# Autodesk Inventor assembly: FullField-ver6-1111-2021
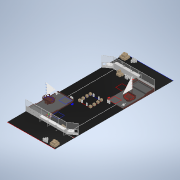
[picture p0: Inventor's stored thumbnail of the model, 180x180]
Saved by Autodesk Inventor 2021 (Build 250183000, 183)
## iProperties
Created: 2021-02-23
Part Number: FullField-ver6-1111-2021
Document SubType Name: Assembly
Designer: CMurray
Author: CMurray
## Documents named in this file (30)
- F:\PHRC CADD 2021\2021 Game Design Challenge\Full Field\Final Assembly\FullField-ver6-1111-2021.iam
- F:\PHRC CADD 2021\2021 Game Design Challenge\Full Field\Parts\FieldFloor-ver1-1111-2021.ipt
- F:\PHRC CADD 2021\2021 Game Design Challenge\Full Field\Parts\Tape\Tape.ipt
- F:\PHRC CADD 2021\2021 Game Design Challenge\Full Field\Parts\Tape\RedAllianceTape-ver1-1111-2021.ipt
- F:\PHRC CADD 2021\2021 Game Design Challenge\Full Field\Parts\Tape\BlueAllianceTape-ver1-1111-2021.ipt
- F:\PHRC CADD 2021\2021 Game Design Challenge\Player Station\Assemblies\DriverStation-ver2-1111-2021.iam
- F:\PHRC CADD 2021\2021 Game Design Challenge\Crow's Nest\Assemblies\CrowsNestFinal-ver3-1111-2021.iam
- F:\PHRC CADD 2021\2021 Game Design Challenge\Main Ship\RedShip-ver1-1111-2021.ipt
- F:\PHRC CADD 2021\2021 Game Design Challenge\Crow's Nest\Parts\Capstan\test.ipt
- F:\PHRC CADD 2021\2021 Game Design Challenge\Crow's Nest\Parts\Capstan\CapTop-ver1-1111-2021.ipt
- F:\PHRC CADD 2021\2021 Game Design Challenge\Crow's Nest\Parts\Capstan\FullSailCapstan-ver2-1111-2021.iam
- F:\PHRC CADD 2021\2021 Game Design Challenge\Full Field\Parts\Tape\Tape2.ipt
- F:\PHRC CADD 2021\2021 Game Design Challenge\Main Ship\BlueShip-ver1-1111-2021.ipt
- F:\PHRC CADD 2021\2021 Game Design Challenge\Crow's Nest\Assemblies\BlueCrowsNestFinal-ver1-1111-2021.iam
- F:\PHRC CADD 2021\2021 Game Design Challenge\Misc\cargoPrototype.ipt
- F:\PHRC CADD 2021\2021 Game Design Challenge\Full Field\Parts\Tape\MidSquareFull.iam
- F:\PHRC CADD 2021\2021 Game Design Challenge\Treasure Chest\PTreasureChestFinal-ver1-1111-2021.ipt
- F:\PHRC CADD 2021\2021 Game Design Challenge\Full Field\Parts\Tape\RedAllianceTape-ver2-1111-2021.ipt
- F:\PHRC CADD 2021\2021 Game Design Challenge\Full Field\Parts\Tape\BlueAllianceTape-ver2-1111-2021.ipt
- F:\PHRC CADD 2021\2021 Game Design Challenge\Anchor\CapstanBottom-ver1-1111-2021.ipt
- F:\PHRC CADD 2021\2021 Game Design Challenge\Anchor\CapstanTop-ver1-1111-2021.ipt
- F:\PHRC CADD 2021\2021 Game Design Challenge\Misc\WaterJug-ver1-1111-2021.ipt
- F:\PHRC CADD 2021\2021 Game Design Challenge\Treasure Chest\BlueMapContainer-ver1-1111-2021.ipt
- F:\PHRC CADD 2021\2021 Game Design Challenge\Treasure Chest\RedMapContainer-ver1-1111-2021.ipt
- F:\PHRC CADD 2021\2021 Game Design Challenge\Full Field\Parts\Tape\ParkingTapeBlueFull.iam
- F:\PHRC CADD 2021\2021 Game Design Challenge\Full Field\Parts\Tape\CrowsNestTapeBlue.ipt
- F:\PHRC CADD 2021\2021 Game Design Challenge\Full Field\Parts\Tape\CrowsNestTapeRed.ipt
- F:\PHRC CADD 2021\2021 Game Design Challenge\Full Field\Parts\Tape\ParkingTapeRedFull.iam
- F:\PHRC CADD 2021\2021 Game Design Challenge\Anchor\CapBottomwChain.iam
- F:\PHRC CADD 2021\2021 Game Design Challenge\Anchor\anchorPlaceholder.ipt
## Components (117 placed, 29 different names)
1. FieldFloor-ver1-1111-2021:1 — Flush:1, Flush:2, Mate:1, Mate:3, Mate:10, Flush:10, Mate:14, Flush:12, Mate:32, Mate:34, Mate:51, Flush:24, Mate:53, Flush:25, Mate:63, Mate:75, Mate:76, Mate:88, Flush:26, Mate:104, Mate:105, Mate:106, Mate:107, Mate:108, Mate:109, Mate:110, Mate:111, Mate:112, Flush:30, Mate:121, Mate:122, Mate:131, Mate:138, Mate:139, Mate:140, Mate:141, Mate:142, Mate:143, Mate:146, Mate:147, Mate:148, Mate:149, Mate:150, Mate:156, Mate:157, Mate:158, Mate:159, Mate:160, Mate:161, Mate:173
2. FieldFloor-ver1-1111-2021:2 — Flush:1, Flush:2, Mate:1, Mate:2, Flush:3, Flush:4, Flush:5, Flush:6, Mate:8, Flush:9, Mate:12, Flush:11, Flush:19, Mate:36, Flush:20, Mate:49, Flush:23, Mate:62, Mate:72, Mate:77, Mate:78, Mate:79, Mate:80, Mate:83, Mate:85, Flush:27, Mate:89, Flush:28, Flush:29, Mate:90, Mate:91, Mate:92, Mate:93, Mate:94, Mate:95, Mate:96, Mate:97, Mate:98, Mate:123, Mate:124, Mate:125, Mate:126, Mate:127, Mate:128, Mate:129, Mate:130, Mate:132, Mate:133, Mate:134, Mate:135, Mate:137, Mate:144, Mate:152, Mate:153, Mate:154, Mate:155, Mate:162, Mate:163, Mate:164, Mate:165, Mate:167
3. WaterJug-ver1-1111-2021:1 — Mate:121
4. WaterJug-ver1-1111-2021:2 — Mate:122
5. WaterJug-ver1-1111-2021:3 — Mate:123
6. WaterJug-ver1-1111-2021:4 — Mate:124
7. WaterJug-ver1-1111-2021:5 — Mate:125
8. WaterJug-ver1-1111-2021:6 — Mate:126
9. WaterJug-ver1-1111-2021:7 — Mate:127
10. WaterJug-ver1-1111-2021:8 — Mate:128
11. WaterJug-ver1-1111-2021:9 — Mate:131
12. WaterJug-ver1-1111-2021:10 — Mate:129
13. WaterJug-ver1-1111-2021:11 — Mate:130
14. cargoPrototype:35 — Mate:137
15. cargoPrototype:36 — Mate:134
16. cargoPrototype:38 — Mate:133
17. cargoPrototype:39 — Mate:135, Mate:151
18. cargoPrototype:40 — Mate:132
19. cargoPrototype:41 — Mate:138
20. cargoPrototype:42 — Mate:142
21. cargoPrototype:43 — Mate:140
22. cargoPrototype:44 — Mate:141
23. cargoPrototype:45 — Mate:139, Mate:145
24. cargoPrototype:46 — Mate:145
25. BlueMapContainer-ver1-1111-2021:1 — Mate:143
26. RedMapContainer-ver1-1111-2021:1 — Mate:144
27. WaterJug-ver1-1111-2021:12 — Mate:146
28. WaterJug-ver1-1111-2021:13 — Mate:150
29. WaterJug-ver1-1111-2021:14 — Mate:147
30. WaterJug-ver1-1111-2021:15 — Mate:149
31. WaterJug-ver1-1111-2021:16 — Mate:148
32. cargoPrototype:47 — Mate:151
33. WaterJug-ver1-1111-2021:17 — Mate:152
34. WaterJug-ver1-1111-2021:18 — Mate:153
35. WaterJug-ver1-1111-2021:19 — Mate:154
36. WaterJug-ver1-1111-2021:20 — Mate:158
37. WaterJug-ver1-1111-2021:21 — Mate:156
38. WaterJug-ver1-1111-2021:22 — Mate:157
39. WaterJug-ver1-1111-2021:23 — Mate:159
40. WaterJug-ver1-1111-2021:24 — Mate:155
41. WaterJug-ver1-1111-2021:25 — Mate:162
42. WaterJug-ver1-1111-2021:26 — Mate:165
43. WaterJug-ver1-1111-2021:27 — Mate:164
44. WaterJug-ver1-1111-2021:28 — Mate:163
45. WaterJug-ver1-1111-2021:29 — Mate:160
46. WaterJug-ver1-1111-2021:30 — Mate:161
47. ParkingTapeBlueFull:1 [sub-assembly] — Mate:166
48. ParkingTapeBlueFull:2 [sub-assembly] — Mate:167
49. CrowsNestTapeBlue:1 — Mate:168, Mate:169
50. CrowsNestTapeRed:1 — Mate:170, Mate:171
51. ParkingTapeRedFull:1 [sub-assembly] — Mate:172
52. ParkingTapeRedFull:2 [sub-assembly] — Mate:173
53. CapBottomwChain:1 [sub-assembly] — Mate:174, Mate:175, Mate:176, Rotational:6
54. anchorPlaceholder:1
55. BlueAllianceTape-ver2-1111-2021:1 — Mate:89, Flush:28, Flush:29
56. RedAllianceTape-ver2-1111-2021:1 — Mate:88, Flush:26, Flush:27
57. MidSquareFull:1 [sub-assembly] — Mate:72, Mate:73, Mate:74
58. Tape2:1 — Mate:49, Flush:23, Mate:50
59. Tape2:2 — Mate:51, Flush:24, Mate:52, Mate:73
60. Tape:1 — Mate:2, Flush:3, Flush:4, Mate:9, Mate:11, Mate:33, Mate:50, Mate:74, Mate:87
61. Tape:2 — Mate:3, Flush:5, Flush:6, Mate:13, Mate:15, Mate:35, Mate:52, Mate:84
62. RedAllianceTape-ver1-1111-2021:1 — Mate:8, Flush:9, Mate:9
63. RedAllianceTape-ver1-1111-2021:2 — Mate:10, Flush:10, Mate:11
64. BlueAllianceTape-ver1-1111-2021:1 — Mate:12, Flush:11, Mate:13
65. BlueAllianceTape-ver1-1111-2021:2 — Mate:14, Flush:12, Mate:15
66. CapstanBottom-ver1-1111-2021:1 — Mate:117, Rotational:5, Flush:31, Flush:32
67. CapstanTop-ver1-1111-2021:1 — Rotational:5
68. CapTop-ver1-1111-2021:2
69. FullSailCapstan-ver2-1111-2021:3 [sub-assembly] — Rotational:4
70. test:2 — Mate:57, Mate:58, Mate:59, Rotational:4
71. BlueShip-ver1-1111-2021:1 — Mate:53, Mate:54, Flush:25, Mate:55, Mate:56, Mate:86, Mate:117, Flush:31, Flush:32
72. BlueCrowsNestFinal-ver1-1111-2021:1 [sub-assembly] — Mate:55, Mate:56, Mate:57, Mate:58, Mate:59, Mate:168, Mate:169
73. CapstanBottom-ver1-1111-2021:2 — Mate:118, Mate:119, Mate:120
74. CapstanTop-ver1-1111-2021:2 — Rotational:6
75. CapTop-ver1-1111-2021:1 — Rotational:2
76. FullSailCapstan-ver2-1111-2021:2 [sub-assembly] — Rotational:1, Rotational:2
77. test:1 — Mate:41, Flush:21, Mate:42, Rotational:1
78. RedShip-ver1-1111-2021:1 — Mate:36, Mate:37, Flush:20, Mate:38, Mate:40, Mate:82, Mate:118, Mate:119, Mate:120, Mate:166, Mate:172, Mate:174, Mate:175, Mate:176
79. CrowsNestFinal-ver3-1111-2021:1 [sub-assembly] — Mate:38, Mate:40, Mate:41, Flush:21, Mate:42, Mate:170, Mate:171
80. DriverStation-ver2-1111-2021:2 [sub-assembly] — Mate:34, Mate:35, Flush:19, Mate:37
81. DriverStation-ver2-1111-2021:1 [sub-assembly] — Mate:32, Mate:33, Mate:54, Flush:30
82. cargoPrototype:9 — Mate:90
83. cargoPrototype:10 — Mate:91
84. cargoPrototype:11 — Mate:92
85. cargoPrototype:12 — Mate:93, Mate:99, Mate:100, Mate:102
86. cargoPrototype:13 — Mate:94, Mate:103
87. cargoPrototype:14 — Mate:95
88. cargoPrototype:15 — Mate:96
89. cargoPrototype:16 — Mate:97, Mate:101
90. cargoPrototype:17 — Mate:98
91. cargoPrototype:18 — Mate:99, Mate:100
92. cargoPrototype:19 — Mate:101
93. cargoPrototype:20 — Mate:102
94. cargoPrototype:21 — Mate:103
95. cargoPrototype:22 — Mate:110
96. cargoPrototype:23 — Mate:112, Mate:113
97. cargoPrototype:24 — Mate:108, Mate:114
98. cargoPrototype:25 — Mate:111
99. cargoPrototype:26 — Mate:107
100. cargoPrototype:27 — Mate:106
101. cargoPrototype:28 — Mate:109
102. cargoPrototype:29 — Mate:105
103. cargoPrototype:30 — Mate:104, Mate:115, Mate:116
104. cargoPrototype:31 — Mate:113
105. cargoPrototype:32 — Mate:114
106. cargoPrototype:33 — Mate:115
107. cargoPrototype:34 — Mate:116
108. cargoPrototype:2 — Mate:63
109. cargoPrototype:3 — Mate:75
110. cargoPrototype:4 — Mate:76
111. cargoPrototype:5 — Mate:78
112. cargoPrototype:6 — Mate:77
113. cargoPrototype:7 — Mate:79
114. cargoPrototype:8 — Mate:80
115. cargoPrototype:1 — Mate:62
116. PTreasureChestFinal-ver1-1111-2021:1 — Mate:82, Mate:83, Mate:84
117. PTreasureChestFinal-ver1-1111-2021:2 — Mate:85, Mate:86, Mate:87
## Relationships (166: Mate 137, Flush 23, RevoluteJoint 6)
- Flush:1: FieldFloor-ver1-1111-2021:1 ↔ FieldFloor-ver1-1111-2021:2
- Flush:2: FieldFloor-ver1-1111-2021:1 ↔ FieldFloor-ver1-1111-2021:2
- Mate:1: FieldFloor-ver1-1111-2021:1 ↔ FieldFloor-ver1-1111-2021:2
- Mate:2: FieldFloor-ver1-1111-2021:2 ↔ Tape:1
- Flush:3: FieldFloor-ver1-1111-2021:2 ↔ Tape:1
- Flush:4 (3606.8 mm): FieldFloor-ver1-1111-2021:2 ↔ Tape:1
- Mate:3: FieldFloor-ver1-1111-2021:1 ↔ Tape:2
- Flush:5: FieldFloor-ver1-1111-2021:2 ↔ Tape:2
- Flush:6 (3606.8 mm): FieldFloor-ver1-1111-2021:2 ↔ Tape:2
- Mate:8: FieldFloor-ver1-1111-2021:2 ↔ RedAllianceTape-ver1-1111-2021:1
- Flush:9: FieldFloor-ver1-1111-2021:2 ↔ RedAllianceTape-ver1-1111-2021:1
- Mate:9: Tape:1 ↔ RedAllianceTape-ver1-1111-2021:1
- Mate:10: FieldFloor-ver1-1111-2021:1 ↔ RedAllianceTape-ver1-1111-2021:2
- Flush:10: FieldFloor-ver1-1111-2021:1 ↔ RedAllianceTape-ver1-1111-2021:2
- Mate:11: Tape:1 ↔ RedAllianceTape-ver1-1111-2021:2
- Mate:12: FieldFloor-ver1-1111-2021:2 ↔ BlueAllianceTape-ver1-1111-2021:1
- Flush:11: FieldFloor-ver1-1111-2021:2 ↔ BlueAllianceTape-ver1-1111-2021:1
- Mate:13: Tape:2 ↔ BlueAllianceTape-ver1-1111-2021:1
- Mate:14: FieldFloor-ver1-1111-2021:1 ↔ BlueAllianceTape-ver1-1111-2021:2
- Flush:12: FieldFloor-ver1-1111-2021:1 ↔ BlueAllianceTape-ver1-1111-2021:2
- Mate:15: Tape:2 ↔ BlueAllianceTape-ver1-1111-2021:2
- Mate:32: FieldFloor-ver1-1111-2021:1 ↔ DriverStation-ver2-1111-2021:1
- Mate:33: Tape:1 ↔ DriverStation-ver2-1111-2021:1
- Mate:34: FieldFloor-ver1-1111-2021:1 ↔ DriverStation-ver2-1111-2021:2
- Mate:35: Tape:2 ↔ DriverStation-ver2-1111-2021:2
- Flush:19: FieldFloor-ver1-1111-2021:2 ↔ DriverStation-ver2-1111-2021:2
- Mate:36: FieldFloor-ver1-1111-2021:2 ↔ RedShip-ver1-1111-2021:1
- Mate:37: RedShip-ver1-1111-2021:1 ↔ DriverStation-ver2-1111-2021:2
- Flush:20: FieldFloor-ver1-1111-2021:2 ↔ RedShip-ver1-1111-2021:1
- Mate:38: RedShip-ver1-1111-2021:1 ↔ CrowsNestFinal-ver3-1111-2021:1
- Mate:40 (1778 mm): RedShip-ver1-1111-2021:1 ↔ CrowsNestFinal-ver3-1111-2021:1
- Mate:41: test:1 ↔ CrowsNestFinal-ver3-1111-2021:1
- Flush:21 (-203.2 mm): test:1 ↔ CrowsNestFinal-ver3-1111-2021:1
- Mate:42 (762 mm): test:1 ↔ CrowsNestFinal-ver3-1111-2021:1
- Rotational:1 [RevoluteJoint]: FullSailCapstan-ver2-1111-2021:2 ↔ test:1
- Rotational:2 [RevoluteJoint]: CapTop-ver1-1111-2021:1 ↔ FullSailCapstan-ver2-1111-2021:2
- Mate:49: FieldFloor-ver1-1111-2021:2 ↔ Tape2:1
- Flush:23 (1524 mm): FieldFloor-ver1-1111-2021:2 ↔ Tape2:1
- Mate:50: Tape2:1 ↔ Tape:1
- Mate:51: FieldFloor-ver1-1111-2021:1 ↔ Tape2:2
- Flush:24 (1524 mm): FieldFloor-ver1-1111-2021:1 ↔ Tape2:2
- Mate:52: Tape2:2 ↔ Tape:2
- Mate:53: FieldFloor-ver1-1111-2021:1 ↔ BlueShip-ver1-1111-2021:1
- Mate:54: BlueShip-ver1-1111-2021:1 ↔ DriverStation-ver2-1111-2021:1
- Flush:25: FieldFloor-ver1-1111-2021:1 ↔ BlueShip-ver1-1111-2021:1
- Mate:55: BlueShip-ver1-1111-2021:1 ↔ BlueCrowsNestFinal-ver1-1111-2021:1
- Mate:56 (1397 mm): BlueShip-ver1-1111-2021:1 ↔ BlueCrowsNestFinal-ver1-1111-2021:1
- Mate:57: test:2 ↔ BlueCrowsNestFinal-ver1-1111-2021:1
- Mate:58 (-203.2 mm): test:2 ↔ BlueCrowsNestFinal-ver1-1111-2021:1
- Mate:59 (762 mm): test:2 ↔ BlueCrowsNestFinal-ver1-1111-2021:1
- [RevoluteJoint]: CapTop-ver1-1111-2021:2 ↔ FullSailCapstan-ver2-1111-2021:3
- Rotational:4 [RevoluteJoint]: FullSailCapstan-ver2-1111-2021:3 ↔ test:2
- Mate:62: FieldFloor-ver1-1111-2021:2 ↔ cargoPrototype:1
- Mate:63: FieldFloor-ver1-1111-2021:1 ↔ cargoPrototype:2
- Mate:72: FieldFloor-ver1-1111-2021:2 ↔ MidSquareFull:1
- Mate:73 (1930.4 mm): MidSquareFull:1 ↔ Tape2:2
- Mate:74 (6553.2 mm): MidSquareFull:1 ↔ Tape:1
- Mate:75: FieldFloor-ver1-1111-2021:1 ↔ cargoPrototype:3
- Mate:76: FieldFloor-ver1-1111-2021:1 ↔ cargoPrototype:4
- Mate:77: FieldFloor-ver1-1111-2021:2 ↔ cargoPrototype:6
- Mate:78: FieldFloor-ver1-1111-2021:2 ↔ cargoPrototype:5
- Mate:79: FieldFloor-ver1-1111-2021:2 ↔ cargoPrototype:7
- Mate:80: FieldFloor-ver1-1111-2021:2 ↔ cargoPrototype:8
- Mate:82 (25.4 mm): RedShip-ver1-1111-2021:1 ↔ PTreasureChestFinal-ver1-1111-2021:1
- Mate:83: FieldFloor-ver1-1111-2021:2 ↔ PTreasureChestFinal-ver1-1111-2021:1
- Mate:84: Tape:2 ↔ PTreasureChestFinal-ver1-1111-2021:1
- Mate:85: FieldFloor-ver1-1111-2021:2 ↔ PTreasureChestFinal-ver1-1111-2021:2
- Mate:86 (25.4 mm): BlueShip-ver1-1111-2021:1 ↔ PTreasureChestFinal-ver1-1111-2021:2
- Mate:87: Tape:1 ↔ PTreasureChestFinal-ver1-1111-2021:2
- Mate:88: FieldFloor-ver1-1111-2021:1 ↔ RedAllianceTape-ver2-1111-2021:1
- Flush:26: FieldFloor-ver1-1111-2021:1 ↔ RedAllianceTape-ver2-1111-2021:1
- Flush:27: FieldFloor-ver1-1111-2021:2 ↔ RedAllianceTape-ver2-1111-2021:1
- Mate:89: FieldFloor-ver1-1111-2021:2 ↔ BlueAllianceTape-ver2-1111-2021:1
- Flush:28: FieldFloor-ver1-1111-2021:2 ↔ BlueAllianceTape-ver2-1111-2021:1
- Flush:29: FieldFloor-ver1-1111-2021:2 ↔ BlueAllianceTape-ver2-1111-2021:1
- Mate:90: FieldFloor-ver1-1111-2021:2 ↔ cargoPrototype:9
- Mate:91: FieldFloor-ver1-1111-2021:2 ↔ cargoPrototype:10
- Mate:92: FieldFloor-ver1-1111-2021:2 ↔ cargoPrototype:11
- Mate:93: FieldFloor-ver1-1111-2021:2 ↔ cargoPrototype:12
- Mate:94: FieldFloor-ver1-1111-2021:2 ↔ cargoPrototype:13
- Mate:95: FieldFloor-ver1-1111-2021:2 ↔ cargoPrototype:14
- Mate:96: FieldFloor-ver1-1111-2021:2 ↔ cargoPrototype:15
- Mate:97: FieldFloor-ver1-1111-2021:2 ↔ cargoPrototype:16
- Mate:98: FieldFloor-ver1-1111-2021:2 ↔ cargoPrototype:17
- Mate:99: cargoPrototype:12 ↔ cargoPrototype:18
- Mate:100: cargoPrototype:12 ↔ cargoPrototype:18
- Mate:101: cargoPrototype:16 ↔ cargoPrototype:19
- Mate:102: cargoPrototype:12 ↔ cargoPrototype:20
- Mate:103: cargoPrototype:13 ↔ cargoPrototype:21
- Mate:104: FieldFloor-ver1-1111-2021:1 ↔ cargoPrototype:30
- Mate:105: FieldFloor-ver1-1111-2021:1 ↔ cargoPrototype:29
- Mate:106: FieldFloor-ver1-1111-2021:1 ↔ cargoPrototype:27
- Mate:107: FieldFloor-ver1-1111-2021:1 ↔ cargoPrototype:26
- Mate:108: FieldFloor-ver1-1111-2021:1 ↔ cargoPrototype:24
- Mate:109: FieldFloor-ver1-1111-2021:1 ↔ cargoPrototype:28
- Mate:110: FieldFloor-ver1-1111-2021:1 ↔ cargoPrototype:22
- Mate:111: FieldFloor-ver1-1111-2021:1 ↔ cargoPrototype:25
- Mate:112: FieldFloor-ver1-1111-2021:1 ↔ cargoPrototype:23
- Mate:113: cargoPrototype:23 ↔ cargoPrototype:31
- Mate:114: cargoPrototype:24 ↔ cargoPrototype:32
- Mate:115: cargoPrototype:30 ↔ cargoPrototype:33
- Mate:116: cargoPrototype:30 ↔ cargoPrototype:34
- Flush:30: FieldFloor-ver1-1111-2021:1 ↔ DriverStation-ver2-1111-2021:1
- Mate:117: CapstanBottom-ver1-1111-2021:1 ↔ BlueShip-ver1-1111-2021:1
- Rotational:5 [RevoluteJoint]: CapstanBottom-ver1-1111-2021:1 ↔ CapstanTop-ver1-1111-2021:1
- Flush:31 (-3937 mm): CapstanBottom-ver1-1111-2021:1 ↔ BlueShip-ver1-1111-2021:1
- Flush:32 (-304.8 mm): CapstanBottom-ver1-1111-2021:1 ↔ BlueShip-ver1-1111-2021:1
- Mate:118: CapstanBottom-ver1-1111-2021:2 ↔ RedShip-ver1-1111-2021:1
- Mate:119 (3937 mm): CapstanBottom-ver1-1111-2021:2 ↔ RedShip-ver1-1111-2021:1
- Mate:120 (304.8 mm): CapstanBottom-ver1-1111-2021:2 ↔ RedShip-ver1-1111-2021:1
- Mate:121: FieldFloor-ver1-1111-2021:1 ↔ WaterJug-ver1-1111-2021:1
- Mate:122: FieldFloor-ver1-1111-2021:1 ↔ WaterJug-ver1-1111-2021:2
- Mate:123: FieldFloor-ver1-1111-2021:2 ↔ WaterJug-ver1-1111-2021:3
- Mate:124: FieldFloor-ver1-1111-2021:2 ↔ WaterJug-ver1-1111-2021:4
- Mate:125: FieldFloor-ver1-1111-2021:2 ↔ WaterJug-ver1-1111-2021:5
- Mate:126: FieldFloor-ver1-1111-2021:2 ↔ WaterJug-ver1-1111-2021:6
- Mate:127: FieldFloor-ver1-1111-2021:2 ↔ WaterJug-ver1-1111-2021:7
- Mate:128: FieldFloor-ver1-1111-2021:2 ↔ WaterJug-ver1-1111-2021:8
- Mate:129: FieldFloor-ver1-1111-2021:2 ↔ WaterJug-ver1-1111-2021:10
- Mate:130: FieldFloor-ver1-1111-2021:2 ↔ WaterJug-ver1-1111-2021:11
- Mate:131: FieldFloor-ver1-1111-2021:1 ↔ WaterJug-ver1-1111-2021:9
- Mate:132: FieldFloor-ver1-1111-2021:2 ↔ cargoPrototype:40
- Mate:133: FieldFloor-ver1-1111-2021:2 ↔ cargoPrototype:38
- Mate:134: FieldFloor-ver1-1111-2021:2 ↔ cargoPrototype:36
- Mate:135: FieldFloor-ver1-1111-2021:2 ↔ cargoPrototype:39
- Mate:137: FieldFloor-ver1-1111-2021:2 ↔ cargoPrototype:35
- Mate:138: FieldFloor-ver1-1111-2021:1 ↔ cargoPrototype:41
- Mate:139: FieldFloor-ver1-1111-2021:1 ↔ cargoPrototype:45
- Mate:140: FieldFloor-ver1-1111-2021:1 ↔ cargoPrototype:43
- Mate:141: FieldFloor-ver1-1111-2021:1 ↔ cargoPrototype:44
- Mate:142: FieldFloor-ver1-1111-2021:1 ↔ cargoPrototype:42
- Mate:143: FieldFloor-ver1-1111-2021:1 ↔ BlueMapContainer-ver1-1111-2021:1
- Mate:144: FieldFloor-ver1-1111-2021:2 ↔ RedMapContainer-ver1-1111-2021:1
- Mate:145: cargoPrototype:45 ↔ cargoPrototype:46
- Mate:146: FieldFloor-ver1-1111-2021:1 ↔ WaterJug-ver1-1111-2021:12
- Mate:147: FieldFloor-ver1-1111-2021:1 ↔ WaterJug-ver1-1111-2021:14
- Mate:148: FieldFloor-ver1-1111-2021:1 ↔ WaterJug-ver1-1111-2021:16
- Mate:149: FieldFloor-ver1-1111-2021:1 ↔ WaterJug-ver1-1111-2021:15
- Mate:150: FieldFloor-ver1-1111-2021:1 ↔ WaterJug-ver1-1111-2021:13
- Mate:151: cargoPrototype:39 ↔ cargoPrototype:47
- Mate:152: FieldFloor-ver1-1111-2021:2 ↔ WaterJug-ver1-1111-2021:17
- Mate:153: FieldFloor-ver1-1111-2021:2 ↔ WaterJug-ver1-1111-2021:18
- Mate:154: FieldFloor-ver1-1111-2021:2 ↔ WaterJug-ver1-1111-2021:19
- Mate:155: FieldFloor-ver1-1111-2021:2 ↔ WaterJug-ver1-1111-2021:24
- Mate:156: FieldFloor-ver1-1111-2021:1 ↔ WaterJug-ver1-1111-2021:21
- Mate:157: FieldFloor-ver1-1111-2021:1 ↔ WaterJug-ver1-1111-2021:22
- Mate:158: FieldFloor-ver1-1111-2021:1 ↔ WaterJug-ver1-1111-2021:20
- Mate:159: FieldFloor-ver1-1111-2021:1 ↔ WaterJug-ver1-1111-2021:23
- Mate:160: FieldFloor-ver1-1111-2021:1 ↔ WaterJug-ver1-1111-2021:29
- Mate:161: FieldFloor-ver1-1111-2021:1 ↔ WaterJug-ver1-1111-2021:30
- Mate:162: FieldFloor-ver1-1111-2021:2 ↔ WaterJug-ver1-1111-2021:25
- Mate:163: FieldFloor-ver1-1111-2021:2 ↔ WaterJug-ver1-1111-2021:28
- Mate:164: FieldFloor-ver1-1111-2021:2 ↔ WaterJug-ver1-1111-2021:27
- Mate:165: FieldFloor-ver1-1111-2021:2 ↔ WaterJug-ver1-1111-2021:26
- Mate:166: ParkingTapeBlueFull:1 ↔ RedShip-ver1-1111-2021:1
- Mate:167: FieldFloor-ver1-1111-2021:2 ↔ ParkingTapeBlueFull:2
- Mate:168: CrowsNestTapeBlue:1 ↔ BlueCrowsNestFinal-ver1-1111-2021:1
- Mate:169: CrowsNestTapeBlue:1 ↔ BlueCrowsNestFinal-ver1-1111-2021:1
- Mate:170: CrowsNestTapeRed:1 ↔ CrowsNestFinal-ver3-1111-2021:1
- Mate:171: CrowsNestTapeRed:1 ↔ CrowsNestFinal-ver3-1111-2021:1
- Mate:172: ParkingTapeRedFull:1 ↔ RedShip-ver1-1111-2021:1
- Mate:173: FieldFloor-ver1-1111-2021:1 ↔ ParkingTapeRedFull:2
- Mate:174: CapBottomwChain:1 ↔ RedShip-ver1-1111-2021:1
- Mate:175 (4064 mm): CapBottomwChain:1 ↔ RedShip-ver1-1111-2021:1
- Mate:176 (304.8 mm): CapBottomwChain:1 ↔ RedShip-ver1-1111-2021:1
- Rotational:6 [RevoluteJoint] (-101.6 mm): CapBottomwChain:1 ↔ CapstanTop-ver1-1111-2021:2
## Named parameters: d150_d121 = 0 mm, d151_d122 = 10.074303 deg
